# Autodesk Inventor assembly: lower_assem
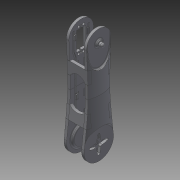
[picture p0: Inventor's stored thumbnail of the model, 180x180]
Saved by Autodesk Inventor 2014 (Build 180170000, 170)
## iProperties
Created: 2014-04-24
Part Number: lower_assem
Document SubType Name: Assembly
Designer: t_emanb
Author: t_emanb
## Documents named in this file (7)
- C:\Users\t_emanb\Documents\3D printed arm\4th version\lower_assem.iam
- C:\Users\t_emanb\Documents\3D printed arm\4th version\lower_curvehorn.ipt
- C:\Users\t_emanb\Documents\3D printed arm\4th version\lower_curvehorn_cable.ipt
- C:\Users\t_emanb\Documents\3D printed arm\4th version\lower_curvepin.ipt
- C:\Users\t_emanb\Documents\3D printed arm\4th version\lower_curveservo.ipt
- C:\Users\t_emanb\Documents\3D printed arm\4th version\lower_bracehorn.ipt
- C:\Users\t_emanb\Documents\3D printed arm\4th version\lower_bracepin.ipt
## Components (8 placed, 6 different names)
1. lower_curvehorn:1 — Flush:2, Mate:4, Mate:7, Mate:11, Mate:21, Mate:23
2. lower_curvehorn_cable:1 — Mate:1, Flush:1, Mate:5, Mate:10, Mate:12, Mate:14, Mate:24
3. lower_curvepin:1 — Mate:1, Flush:1, Mate:17, Mate:18, Mate:20, Angle:1, Mate:22, Mate:24, Mate:25, Mate:26
4. lower_curveservo:1 — Flush:2, Mate:4, Angle:1, Mate:23
5. lower_bracehorn:1 — Mate:5, Mate:7, Mate:10, Mate:11
6. lower_bracehorn:2 — Mate:12, Mate:14, Mate:21
7. lower_bracepin:1 — Mate:17, Mate:25, Mate:26
8. lower_bracepin:2 — Mate:18, Mate:20, Mate:22
## Relationships (20: Mate 17, Flush 2, Angle 1)
- Mate:1: lower_curvehorn_cable:1 ↔ lower_curvepin:1
- Flush:1: lower_curvehorn_cable:1 ↔ lower_curvepin:1
- Flush:2: lower_curvehorn:1 ↔ lower_curveservo:1
- Mate:4: lower_curvehorn:1 ↔ lower_curveservo:1
- Mate:5: lower_curvehorn_cable:1 ↔ lower_bracehorn:1
- Mate:7: lower_curvehorn:1 ↔ lower_bracehorn:1
- Mate:10: lower_curvehorn_cable:1 ↔ lower_bracehorn:1
- Mate:11: lower_curvehorn:1 ↔ lower_bracehorn:1
- Mate:12: lower_curvehorn_cable:1 ↔ lower_bracehorn:2
- Mate:14: lower_curvehorn_cable:1 ↔ lower_bracehorn:2
- Mate:17: lower_curvepin:1 ↔ lower_bracepin:1
- Mate:18: lower_curvepin:1 ↔ lower_bracepin:2
- Mate:20: lower_curvepin:1 ↔ lower_bracepin:2
- Angle:1 (180 deg): lower_curvepin:1 ↔ lower_curveservo:1
- Mate:21: lower_curvehorn:1 ↔ lower_bracehorn:2
- Mate:22: lower_curvepin:1 ↔ lower_bracepin:2
- Mate:23: lower_curvehorn:1 ↔ lower_curveservo:1
- Mate:24: lower_curvehorn_cable:1 ↔ lower_curvepin:1
- Mate:25: lower_curvepin:1 ↔ lower_bracepin:1
- Mate:26: lower_curvepin:1 ↔ lower_bracepin:1
